# Autodesk Inventor assembly: InnerFrameInternals
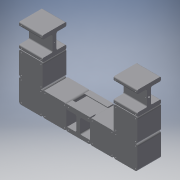
[picture p0: Inventor's stored thumbnail of the model, 180x180]
Saved by Autodesk Inventor 2016 (Build 200138000, 138)
## iProperties
Created: 2016-05-22
Part Number: InnerFrameInternals
Document SubType Name: Assembly
Designer: Kurtis
Author: Kurtis
## Documents named in this file (5)
- C:\Users\Kurtis\Git\CAD\Sentry Camera\cad\InnerFrameInternals.iam
- C:\Users\Kurtis\Git\CAD\Sentry Camera\cad\60x60CameraMount.ipt
- C:\Users\Kurtis\Git\CAD\Sentry Camera\cad\60x60Spacer.ipt
- C:\Users\Kurtis\Git\CAD\Sentry Camera\cad\60x60Idler.ipt
- C:\Users\Kurtis\Git\CAD\Sentry Camera\cad\60x60IdlerNoMotor.ipt
## Components (9 placed, 4 different names)
1. 60x60CameraMount:1 — Mate:1, Flush:1, Flush:2, Flush:3, Mate:2, Flush:4
2. 60x60Spacer:1 — Flush:3, Mate:2, Flush:4, Mate:5, Flush:9, Flush:10
3. 60x60Spacer:2 — Flush:11, Flush:12, Mate:6, Flush:15, Flush:16, Mate:8
4. 60x60Spacer:3 — Mate:1, Flush:1, Flush:2, Flush:5, Mate:3, Flush:6
5. 60x60Spacer:4 — Flush:5, Mate:3, Flush:6, Flush:7, Flush:8, Mate:4
6. 60x60Spacer:5 — Flush:7, Flush:8, Mate:4, Flush:13, Flush:14, Mate:7
7. 60x60Spacer:6 — Mate:5, Flush:9, Flush:10, Flush:11, Flush:12, Mate:6
8. 60x60Idler:1 — Flush:13, Flush:14, Mate:7
9. 60x60IdlerNoMotor:1 — Flush:15, Flush:16, Mate:8
## Relationships (24: Flush 16, Mate 8)
- Mate:1: 60x60CameraMount:1 ↔ 60x60Spacer:3
- Flush:1: 60x60CameraMount:1 ↔ 60x60Spacer:3
- Flush:2: 60x60CameraMount:1 ↔ 60x60Spacer:3
- Flush:3: 60x60CameraMount:1 ↔ 60x60Spacer:1
- Mate:2: 60x60CameraMount:1 ↔ 60x60Spacer:1
- Flush:4: 60x60CameraMount:1 ↔ 60x60Spacer:1
- Flush:5: 60x60Spacer:3 ↔ 60x60Spacer:4
- Mate:3: 60x60Spacer:3 ↔ 60x60Spacer:4
- Flush:6: 60x60Spacer:3 ↔ 60x60Spacer:4
- Flush:7: 60x60Spacer:4 ↔ 60x60Spacer:5
- Flush:8: 60x60Spacer:4 ↔ 60x60Spacer:5
- Mate:4: 60x60Spacer:4 ↔ 60x60Spacer:5
- Mate:5: 60x60Spacer:1 ↔ 60x60Spacer:6
- Flush:9: 60x60Spacer:1 ↔ 60x60Spacer:6
- Flush:10: 60x60Spacer:1 ↔ 60x60Spacer:6
- Flush:11: 60x60Spacer:2 ↔ 60x60Spacer:6
- Flush:12: 60x60Spacer:2 ↔ 60x60Spacer:6
- Mate:6: 60x60Spacer:2 ↔ 60x60Spacer:6
- Flush:13: 60x60Spacer:5 ↔ 60x60Idler:1
- Flush:14: 60x60Spacer:5 ↔ 60x60Idler:1
- Mate:7: 60x60Spacer:5 ↔ 60x60Idler:1
- Flush:15: 60x60Spacer:2 ↔ 60x60IdlerNoMotor:1
- Flush:16: 60x60Spacer:2 ↔ 60x60IdlerNoMotor:1
- Mate:8: 60x60Spacer:2 ↔ 60x60IdlerNoMotor:1
